# Autodesk Inventor assembly: Shaft
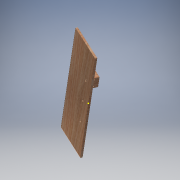
[picture p0: Inventor's stored thumbnail of the model, 180x180]
Saved by Autodesk Inventor 2016 (Build 200138000, 138)
## iProperties
Created: 2016-04-01
Part Number: Shaft
Document SubType Name: Assembly
Designer: mkepler
Author: mkepler
## Documents named in this file (7)
- C:\Users\mkepler\Google Drive\Michael Kepler\College\ECE\ECE 590\Project 2\Physical Design\Inventor Files\Shaft\Shaft.iam
- C:\Users\mkepler\Google Drive\Michael Kepler\College\ECE\ECE 590\Project 2\Physical Design\Inventor Files\Shaft\Base.ipt
- C:\Users\mkepler\Google Drive\Michael Kepler\College\ECE\ECE 590\Project 2\Physical Design\Inventor Files\xl320Servo.ipt
- C:\Users\mkepler\Google Drive\Michael Kepler\College\ECE\ECE 590\Project 2\Physical Design\Inventor Files\Shaft\RotatorBottom.ipt
- C:\Users\mkepler\Google Drive\Michael Kepler\College\ECE\ECE 590\Project 2\Physical Design\Inventor Files\Shaft\SideSupport.ipt
- C:\Users\mkepler\Google Drive\Michael Kepler\College\ECE\ECE 590\Project 2\Physical Design\Inventor Files\Shaft\FrontSupport.ipt
- C:\Users\mkepler\Google Drive\Michael Kepler\College\ECE\ECE 590\Project 2\Physical Design\Inventor Files\Shaft\FrontSupportCover.ipt
## Components (7 placed, 6 different names)
1. Base:1 — Insert:1, Insert:2, Insert:7, Insert:8, Insert:9, Insert:10, Insert:11, Insert:12
2. xl320Servo:1 — Insert:1, Insert:2, Insert:3, Insert:4
3. RotatorBottom:1 — Insert:3, Insert:4
4. SideSupport:1 — Insert:7, Insert:8
5. SideSupport:2 — Insert:9, Insert:10, Insert:13, Insert:14
6. FrontSupport:1 — Insert:11, Insert:12
7. FrontSupportCover:1 — Insert:13, Insert:14
## Relationships (12: Insert 12)
- Insert:1: Base:1 ↔ xl320Servo:1
- Insert:2: Base:1 ↔ xl320Servo:1
- Insert:3: xl320Servo:1 ↔ RotatorBottom:1
- Insert:4: xl320Servo:1 ↔ RotatorBottom:1
- Insert:7: Base:1 ↔ SideSupport:1
- Insert:8: Base:1 ↔ SideSupport:1
- Insert:9: Base:1 ↔ SideSupport:2
- Insert:10: Base:1 ↔ SideSupport:2
- Insert:11: Base:1 ↔ FrontSupport:1
- Insert:12: Base:1 ↔ FrontSupport:1
- Insert:13: SideSupport:2 ↔ FrontSupportCover:1
- Insert:14: SideSupport:2 ↔ FrontSupportCover:1
